# Autodesk Inventor assembly: assembly
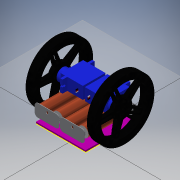
[picture p0: Inventor's stored thumbnail of the model, 180x180]
Saved by Autodesk Inventor 2016 (Build 200138000, 138)
## iProperties
Created: 2016-01-12
Part Number: assembly
Document SubType Name: Assembly
Designer: jferner
Author: jferner
## Documents named in this file (6)
- C:\dev\minirobot\mechanical\assembly.iam
- C:\dev\minirobot\mechanical\micro-servo.ipt
- C:\dev\minirobot\mechanical\wheel.ipt
- C:\dev\minirobot\mechanical\battery-aaa.ipt
- C:\dev\minirobot\mechanical\assembly-pcb.iam
- C:\dev\minirobot\mechanical\BK-5003-ND.ipt
## Components (13 placed, 5 different names)
1. micro-servo:1 — Mate:1, Flush:1, Flush:2, Mate:2, Insert:2, Mate:3, Mate:6, Flush:9, Flush:10
2. micro-servo:2 — Mate:1, Flush:1, Flush:2, Insert:1, Mate:8, Flush:13
3. wheel:1 — Insert:2
4. wheel:2 — Insert:1
5. battery-aaa:1 — Insert:5, Insert:9
6. battery-aaa:2 — Insert:4, Insert:7
7. battery-aaa:3 — Mate:7, Insert:3, Insert:10
8. battery-aaa:4 — Insert:6, Insert:8
9. assembly-pcb:1 [sub-assembly] — Mate:6, Flush:9, Flush:10
10. BK-5003-ND:1 — Insert:7, Insert:10
11. BK-5003-ND:2 — Insert:5, Insert:6
12. BK-5003-ND:3 — Insert:8, Insert:9, Flush:11, Flush:12, Mate:9
13. BK-5003-ND:4 — Mate:7, Insert:3, Insert:4, Flush:11, Flush:12, Mate:8, Mate:9, Flush:13
## Relationships (24: Insert 10, Mate 7, Flush 7)
- Mate:1 (2 mm): micro-servo:1 ↔ micro-servo:2
- Flush:1: micro-servo:1 ↔ micro-servo:2
- Flush:2: micro-servo:1 ↔ micro-servo:2
- Mate:2: micro-servo:1
- Insert:1: micro-servo:2 ↔ wheel:2
- Insert:2: micro-servo:1 ↔ wheel:1
- Mate:3: micro-servo:1
- Mate:6 (-24 mm): micro-servo:1 ↔ assembly-pcb:1
- Flush:9 (4 mm): micro-servo:1 ↔ assembly-pcb:1
- Flush:10 (21 mm): micro-servo:1 ↔ assembly-pcb:1
- Mate:7: battery-aaa:3 ↔ BK-5003-ND:4
- Insert:3: battery-aaa:3 ↔ BK-5003-ND:4
- Insert:4 (3.81 mm): battery-aaa:2 ↔ BK-5003-ND:4
- Insert:5: battery-aaa:1 ↔ BK-5003-ND:2
- Insert:6 (3.81 mm): battery-aaa:4 ↔ BK-5003-ND:2
- Insert:7: battery-aaa:2 ↔ BK-5003-ND:1
- Insert:8: battery-aaa:4 ↔ BK-5003-ND:3
- Insert:9 (3.81 mm): battery-aaa:1 ↔ BK-5003-ND:3
- Insert:10 (3.81 mm): battery-aaa:3 ↔ BK-5003-ND:1
- Flush:11: BK-5003-ND:3 ↔ BK-5003-ND:4
- Flush:12: BK-5003-ND:3 ↔ BK-5003-ND:4
- Mate:8 (1 mm): micro-servo:2 ↔ BK-5003-ND:4
- Mate:9 (1 mm): BK-5003-ND:3 ↔ BK-5003-ND:4
- Flush:13 (0.5 mm): micro-servo:2 ↔ BK-5003-ND:4
## Named parameters: compressedCoilLength = 3.81 mm
